# Autodesk Inventor assembly: TOF Assembly
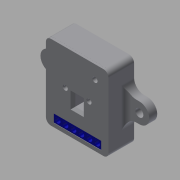
[picture p0: Inventor's stored thumbnail of the model, 180x180]
Saved by Autodesk Inventor 2019.3 (Build 233278000, 278)
## iProperties
Created: 2019-02-11
Part Number: TOF Assembly
Document SubType Name: Assembly
Designer: erics
Mass: 19.2136 g
Surface Area: 241.537 cm^2
Volume: 19.2136 cm^3
Density: 1 g/cm^3
Author: erics
## Documents named in this file (5)
- D:\Users\erics\Documents\CAN TOF\CAD\TOF Assembly.iam
- D:\Users\erics\Documents\CAN TOF\CAD\CAN TOF\CAN TOF.iam
- D:\Users\erics\Documents\CAD Library\Electronics\Adafruit VL53L0X.ipt
- D:\Users\erics\Documents\CAN TOF\CAD\TOF Case P1.ipt
- D:\Users\erics\Documents\CAN TOF\CAD\TOF Case P2_ISO.ipt
## Components (4 placed, 4 different names)
1. CAN TOF:1 [sub-assembly] — Mate:1, Mate:2, Mate:3, Mate:4, Mate:5, Mate:6
2. Adafruit VL53L0X:1 — Mate:1, Mate:2, Mate:3
3. TOF Case P1:1 — Mate:4, Mate:5, Mate:6, Flush:1, Flush:2, Mate:7
4. TOF Case P2_ISO:1 — Flush:1, Flush:2, Mate:7
## Relationships (9: Mate 7, Flush 2)
- Mate:1: CAN TOF:1 ↔ Adafruit VL53L0X:1
- Mate:2: CAN TOF:1 ↔ Adafruit VL53L0X:1
- Mate:3: CAN TOF:1 ↔ Adafruit VL53L0X:1
- Mate:4: CAN TOF:1 ↔ TOF Case P1:1
- Mate:5: CAN TOF:1 ↔ TOF Case P1:1
- Mate:6: CAN TOF:1 ↔ TOF Case P1:1
- Flush:1: TOF Case P1:1 ↔ TOF Case P2_ISO:1
- Flush:2: TOF Case P1:1 ↔ TOF Case P2_ISO:1
- Mate:7: TOF Case P1:1 ↔ TOF Case P2_ISO:1
